# Autodesk Inventor assembly: Shooter
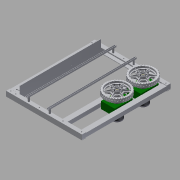
[picture p0: Inventor's stored thumbnail of the model, 180x180]
Saved by Autodesk Inventor 2013 (Build 170138000, 138)
## iProperties
Created: 2013-01-27
Part Number: Shooter
Document SubType Name: Assembly
Designer: Naphat
Author: Naphat
## Documents named in this file (12)
- C:\Autodesk\gruntmaster6000-cad\Shooter\Shooter.iam
- C:\Autodesk\gruntmaster6000-cad\Imported Components\Wheels\Basic Wheel\Shooter Basic Design.iam
- C:\Autodesk\gruntmaster6000-cad\Shooter\Shooter Pressure Channel.ipt
- C:\Autodesk\gruntmaster6000-cad\Shooter\Low Friction Frisbee Track.ipt
- C:\Autodesk\gruntmaster6000-cad\Shooter\Shooter Frame - Rear.ipt
- C:\Autodesk\gruntmaster6000-cad\Shooter\Shooter Frame - Left.ipt
- C:\Autodesk\gruntmaster6000-cad\Shooter\Shooter Frame - Right.ipt
- C:\Autodesk\gruntmaster6000-cad\Shooter\Shooter Frame - Front.ipt
- C:\Autodesk\gruntmaster6000-cad\Shooter\Shooter Frame - CIM Mount.ipt
- C:\Autodesk\gruntmaster6000-cad\Shooter\Shooter Frame - Firing Pin Mount.ipt
- C:\Autodesk\gruntmaster6000-cad\Frisbee.ipt
- C:\Autodesk\gruntmaster6000-cad\Prototypes\Shooter Firing Pin\.25in x 1 in Spacer.ipt
## Components (17 placed, 12 different names)
1. Pressure Channel — Mate:212, Mate:213, Mate:230, Flush:4
2. Low Friction Frisbee Track:1 — Mate:219, Mate:231
3. Low Friction Frisbee Track:2 — Mate:218, Mate:232, Mate:233
4. Frisbee:2 — Mate:230
5. .25in x 1 in Spacer:1 — Mate:238, Mate:239
6. .25in x 1 in Spacer:2 — Mate:240, Mate:241
7. .25in x 1 in Spacer:3 — Mate:234, Mate:235
8. .25in x 1 in Spacer:4 — Mate:236, Mate:237
9. Wheel Assy:Rear [sub-assembly] — Flush:3, Insert:7, Insert:8
10. Wheel Assy:Front [sub-assembly] — Flush:3, Insert:9, Insert:10
11. Shooter Frame - Firing Pin Mount:1 — Mate:223, Mate:224, Insert:11, Insert:12
12. Shooter Frame - Rear:1 — Insert:2, Insert:4, Insert:6, Mate:213, Mate:218, Mate:219, Insert:11, Mate:231, Mate:233, Mate:234, Mate:235, Mate:236, Mate:237
13. Shooter Frame - Front:1 — Insert:1, Insert:3, Insert:5, Mate:214, Mate:215, Mate:223, Mate:224, Insert:12, Mate:232, Mate:238, Mate:239, Mate:240, Mate:241
14. Shooter Frame - Right:1 — Insert:1, Insert:2, Insert:7, Insert:8, Insert:9, Insert:10
15. Shooter Frame - CIM Mount:1 — Insert:3, Insert:4
16. Shooter Frame - Left:1 — Insert:5, Insert:6, Mate:212, Mate:216
17. Shooter Frame - Left:2 — Mate:214, Mate:215, Mate:216, Flush:4
## Relationships (35: Mate 21, Insert 12, Flush 2)
- Flush:3: Wheel Assy:Rear ↔ Wheel Assy:Front
- Insert:1: Shooter Frame - Front:1 ↔ Shooter Frame - Right:1
- Insert:2: Shooter Frame - Rear:1 ↔ Shooter Frame - Right:1
- Insert:3: Shooter Frame - Front:1 ↔ Shooter Frame - CIM Mount:1
- Insert:4: Shooter Frame - Rear:1 ↔ Shooter Frame - CIM Mount:1
- Insert:5: Shooter Frame - Front:1 ↔ Shooter Frame - Left:1
- Insert:6: Shooter Frame - Rear:1 ↔ Shooter Frame - Left:1
- Mate:212: Pressure Channel ↔ Shooter Frame - Left:1
- Mate:213: Pressure Channel ↔ Shooter Frame - Rear:1
- Mate:214: Shooter Frame - Front:1 ↔ Shooter Frame - Left:2
- Mate:215: Shooter Frame - Front:1 ↔ Shooter Frame - Left:2
- Mate:216: Shooter Frame - Left:1 ↔ Shooter Frame - Left:2
- Mate:218 (25.4 mm): Low Friction Frisbee Track:2 ↔ Shooter Frame - Rear:1
- Mate:219 (25.4 mm): Low Friction Frisbee Track:1 ↔ Shooter Frame - Rear:1
- Insert:7: Wheel Assy:Rear ↔ Shooter Frame - Right:1
- Insert:8: Wheel Assy:Rear ↔ Shooter Frame - Right:1
- Insert:9: Wheel Assy:Front ↔ Shooter Frame - Right:1
- Insert:10: Wheel Assy:Front ↔ Shooter Frame - Right:1
- Mate:223: Shooter Frame - Firing Pin Mount:1 ↔ Shooter Frame - Front:1
- Mate:224: Shooter Frame - Firing Pin Mount:1 ↔ Shooter Frame - Front:1
- Insert:11: Shooter Frame - Firing Pin Mount:1 ↔ Shooter Frame - Rear:1
- Insert:12: Shooter Frame - Firing Pin Mount:1 ↔ Shooter Frame - Front:1
- Mate:230: Pressure Channel ↔ Frisbee:2
- Flush:4: Pressure Channel ↔ Shooter Frame - Left:2
- Mate:231: Low Friction Frisbee Track:1 ↔ Shooter Frame - Rear:1
- Mate:232: Low Friction Frisbee Track:2 ↔ Shooter Frame - Front:1
- Mate:233: Low Friction Frisbee Track:2 ↔ Shooter Frame - Rear:1
- Mate:234: .25in x 1 in Spacer:3 ↔ Shooter Frame - Rear:1
- Mate:235: .25in x 1 in Spacer:3 ↔ Shooter Frame - Rear:1
- Mate:236: .25in x 1 in Spacer:4 ↔ Shooter Frame - Rear:1
- Mate:237: .25in x 1 in Spacer:4 ↔ Shooter Frame - Rear:1
- Mate:238: .25in x 1 in Spacer:1 ↔ Shooter Frame - Front:1
- Mate:239: .25in x 1 in Spacer:1 ↔ Shooter Frame - Front:1
- Mate:240: .25in x 1 in Spacer:2 ↔ Shooter Frame - Front:1
- Mate:241: .25in x 1 in Spacer:2 ↔ Shooter Frame - Front:1
